# Autodesk Inventor assembly: Hand Assembly
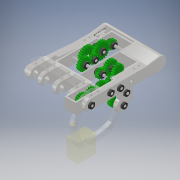
[picture p0: Inventor's stored thumbnail of the model, 180x180]
Saved by Autodesk Inventor 2017 (Build 210142000, 142)
## iProperties
Created: 2016-09-28
Part Number: Hand Assembly
Document SubType Name: Assembly
Designer: cmcdona
Author: cmcdona
## Documents named in this file (25)
- C:\Users\Sam\Desktop\1C03-20171130T033242Z-001\1C03\Project Files Final I Hope Maybe Not Probably Not\Hand Assembly.iam
- C:\Users\Sam\Desktop\1C03-20171130T033242Z-001\1C03\Project Files Final I Hope Maybe Not Probably Not\Hand - Frame.ipt
- C:\Users\Sam\Desktop\1C03-20171130T033242Z-001\1C03\Project Files Final I Hope Maybe Not Probably Not\Hand - Digit 4.ipt
- C:\Users\Sam\Desktop\1C03-20171130T033242Z-001\1C03\Project Files Final I Hope Maybe Not Probably Not\Hand - Digit 0-1.ipt
- C:\Users\Sam\Desktop\1C03-20171130T033242Z-001\1C03\Project Files Final I Hope Maybe Not Probably Not\Hand - Distal Bridge.ipt
- C:\Users\Sam\Desktop\1C03-20171130T033242Z-001\1C03\Project Files Final I Hope Maybe Not Probably Not\Hand - Digit 2-3.ipt
- C:\Users\Sam\Desktop\1C03-20171130T033242Z-001\1C03\Project Files Final I Hope Maybe Not Probably Not\Hand - Proximal Bridge.ipt
- C:\Users\Sam\Desktop\1C03-20171130T033242Z-001\1C03\Project Files Final I Hope Maybe Not Probably Not\Hand - Functional Workspace.ipt
- C:\Users\Sam\Desktop\1C03-20171130T033242Z-001\1C03\Project Files Final I Hope Maybe Not Probably Not\Input Motor.ipt
- C:\Users\Sam\Desktop\1C03-20171130T033242Z-001\1C03\Project Files\GIVEN PARTS\THREADED STUDS\91565A838_STEEL THREADED ROD.ipt
- C:\Users\Sam\Desktop\1C03-20171130T033242Z-001\1C03\Project Files\GIVEN PARTS\NUTS\90480A009_STEEL HEX NUT.ipt
- C:\Users\Sam\Desktop\1C03-20171130T033242Z-001\1C03\Project Files Final I Hope Maybe Not Probably Not\Hand Assembly\Design Accelerator\Spur Gears1.iam
- C:\Users\Sam\Desktop\1C03-20171130T033242Z-001\1C03\Project Files Final I Hope Maybe Not Probably Not\Hand Assembly\Design Accelerator\Spur Gears2.iam
- C:\Users\Sam\Desktop\1C03-20171130T033242Z-001\1C03\Project Files Final I Hope Maybe Not Probably Not\Hand Assembly\Design Accelerator\Spur Gear12.ipt
- C:\Users\Sam\Desktop\1C03-20171130T033242Z-001\1C03\Project Files\GIVEN PARTS\THREADED STUDS\91565A838_STEEL THREADED ROD FULL.ipt
- C:\Users\Sam\Desktop\1C03-20171130T033242Z-001\1C03\Project Files Final I Hope Maybe Not Probably Not\Hand Assembly\Design Accelerator\Spur Gears3.iam
- C:\Users\Sam\Desktop\1C03-20171130T033242Z-001\1C03\Project Files Final I Hope Maybe Not Probably Not\Hand Assembly\Design Accelerator\Spur Gears4.iam
- C:\Users\Sam\Desktop\1C03-20171130T033242Z-001\1C03\Project Files Final I Hope Maybe Not Probably Not\Hand Assembly\Design Accelerator\Spur Gears5.iam
- C:\Users\Sam\Desktop\1C03-20171130T033242Z-001\1C03\Project Files Final I Hope Maybe Not Probably Not\Midsection.ipt
- C:\Users\Sam\Desktop\1C03-20171130T033242Z-001\1C03\Project Files\GIVEN PARTS\THREADED STUDS\91565A838_STEEL THREADED ROD HALF.ipt
- C:\Users\Sam\Desktop\1C03-20171130T033242Z-001\1C03\Project Files Final I Hope Maybe Not Probably Not\Hand Assembly\Design Accelerator\Spur Gears6.iam
- C:\Users\Sam\Desktop\1C03-20171130T033242Z-001\1C03\Project Files\GIVEN PARTS\THREADED STUDS\91565A838_STEEL THREADED ROD FINAL.ipt
- C:\Users\Sam\Desktop\1C03-20171130T033242Z-001\1C03\Project Files Final I Hope Maybe Not Probably Not\Hand Assembly\Design Accelerator\Spur Gears7.iam
- C:\Users\Sam\Desktop\1C03-20171130T033242Z-001\1C03\Project Files\GIVEN PARTS\THREADED STUDS\Finger.ipt
- C:\Users\Sam\Desktop\Inventor Files\Version I\SENGH IS KENGH.ipt
## Components (58 placed, 18 different names)
1. SENGH IS KENGH:1 — Flush:45
2. Midsection:1 — Mate:68, Mate:69, Mate:70, Flush:41, Mate:75, Mate:83, Flush:45
3. Finger:4 — Mate:99, Flush:44
4. Finger:3 — Mate:96, Mate:98, Mate:99, Flush:44
5. Finger:2 — Flush:43, Mate:95
6. Finger:1 — Mate:89, Mate:91, Mate:93, Flush:43
7. Input Motor:1 — Mate:22, Mate:23, Mate:48, Mate:49, Mate:51
8. Hand - Functional Workspace:1 — Mate:19, Mate:20, Mate:21
9. Hand - Proximal Bridge:1 — Mate:16, Mate:17, Mate:18
10. Hand - Digit 2-3:3 — Mate:13, Mate:14, Mate:15, Mate:24, Mate:28
11. Hand - Digit 2-3:2 — Mate:10, Mate:11, Mate:12, Mate:69
12. Hand - Digit 2-3:1 — Mate:7, Mate:8, Mate:9
13. Hand - Distal Bridge:1 — Mate:4, Mate:5, Mate:6, Mate:7, Mate:8, Mate:9, Mate:10, Mate:11, Mate:12, Mate:13, Mate:14, Mate:15
14. Hand - Digit 0-1:1 — Mate:2, Flush:3, Mate:3, Mate:6, Mate:19, Mate:20, Mate:21, Mate:26, Mate:29, Mate:31, Mate:33, Mate:98
15. Hand - Digit 4:1 — Flush:1, Flush:2, Mate:1, Mate:4, Mate:5
16. Hand - Frame:1 — Flush:1, Flush:2, Mate:1, Mate:2, Flush:3, Mate:3, Mate:16, Mate:17, Mate:18, Mate:22, Mate:23, Mate:65, Mate:68, Mate:70, Flush:41, Mate:72, Mate:85
17. Spur Gears:4 [sub-assembly] — Mate:50, Mate:51, Mate:54, Mate:55, Mate:56, Mate:57, Mate:61
18. Spur Gears:5 [sub-assembly] — Mate:60, Mate:61, Mate:62, Mate:64, Mate:73
19. Spur Gears:6 [sub-assembly] — Mate:66, Mate:67, Mate:71, Insert:6, Insert:7
20. Spur Gear1:1 — Mate:34, Flush:8
21. Spur Gears:3 [sub-assembly] — Flush:39, Mate:39, Mate:40, Mate:43, Mate:44, Mate:45, Mate:46, Mate:86
22. Spur Gears:2 [sub-assembly] — Mate:32, Mate:33, Flush:8, Mate:40, Mate:41, Mate:42
23. Spur Gears:1 [sub-assembly] — Mate:27, Mate:28, Flush:39, Mate:39, Mate:91
24. Spur Gears:7 [sub-assembly] — Mate:74, Mate:75, Mate:77, Mate:79, Mate:81, Insert:8, Insert:9
25. Spur Gears:8 [sub-assembly] — Mate:84, Mate:85, Mate:86, Mate:87
26. 91565A838_STEEL THREADED ROD FULL:2 — Mate:48, Mate:49, Mate:50, Mate:52, Mate:53
27. 91565A838_STEEL THREADED ROD HALF:1 — Mate:71, Mate:72, Mate:74, Mate:76, Mate:78
28. 91565A838_STEEL THREADED ROD FINAL:1 — Mate:81, Mate:83, Mate:84, Mate:88
29. 91565A838_STEEL THREADED ROD:4 — Mate:44, Insert:11
30. 91565A838_STEEL THREADED ROD:1 — Mate:24, Mate:25, Flush:4, Mate:27, Insert:13, Mate:90
31. 91565A838_STEEL THREADED ROD:2 — Mate:29, Flush:6, Mate:30, Mate:32, Mate:34, Insert:2, Mate:97
32. 91565A838_STEEL THREADED ROD:3 — Insert:1, Mate:42, Insert:12
33. 91565A838_STEEL THREADED ROD:7 — Mate:45, Mate:47, Flush:42, Insert:10
34. 91565A838_STEEL THREADED ROD:5 — Mate:56, Insert:4, Mate:58, Mate:60
35. 91565A838_STEEL THREADED ROD:6 — Mate:64, Mate:65, Mate:66
36. 90480A009_STEEL HEX NUT:2 — Flush:7, Mate:30, Mate:31
37. 90480A009_STEEL HEX NUT:21 — Insert:12
38. 90480A009_STEEL HEX NUT:1 — Mate:25, Flush:5, Mate:26
39. 90480A009_STEEL HEX NUT:3 — Insert:2
40. 90480A009_STEEL HEX NUT:4 — Insert:1, Mate:41
41. 90480A009_STEEL HEX NUT:5 — Mate:46, Mate:47, Flush:42
42. 90480A009_STEEL HEX NUT:6 — Mate:43
43. 90480A009_STEEL HEX NUT:7 — Mate:52, Mate:55
44. 90480A009_STEEL HEX NUT:8 — Mate:53, Mate:54
45. 90480A009_STEEL HEX NUT:9 — Insert:4, Mate:57
46. 90480A009_STEEL HEX NUT:10 — Mate:58, Mate:62
47. 90480A009_STEEL HEX NUT:12 — Mate:73
48. 90480A009_STEEL HEX NUT:11 — Mate:67
49. 90480A009_STEEL HEX NUT:13 — Insert:6
50. 90480A009_STEEL HEX NUT:14 — Insert:7
51. 90480A009_STEEL HEX NUT:15 — Mate:76, Mate:77
52. 90480A009_STEEL HEX NUT:16 — Mate:78, Mate:79
53. 90480A009_STEEL HEX NUT:17 — Insert:8
54. 90480A009_STEEL HEX NUT:18 — Insert:9
55. 90480A009_STEEL HEX NUT:19 — Mate:87, Mate:88
56. 90480A009_STEEL HEX NUT:20 — Insert:10
57. 90480A009_STEEL HEX NUT:22 — Insert:11
58. 90480A009_STEEL HEX NUT:23 — Insert:13
## Relationships (118: Mate 91, Flush 14, Insert 13)
- Flush:1: Hand - Digit 4:1 ↔ Hand - Frame:1
- Flush:2: Hand - Digit 4:1 ↔ Hand - Frame:1
- Mate:1: Hand - Digit 4:1 ↔ Hand - Frame:1
- Mate:2: Hand - Digit 0-1:1 ↔ Hand - Frame:1
- Flush:3: Hand - Digit 0-1:1 ↔ Hand - Frame:1
- Mate:3: Hand - Digit 0-1:1 ↔ Hand - Frame:1
- Mate:4: Hand - Distal Bridge:1 ↔ Hand - Digit 4:1
- Mate:5: Hand - Distal Bridge:1 ↔ Hand - Digit 4:1
- Mate:6: Hand - Distal Bridge:1 ↔ Hand - Digit 0-1:1
- Mate:7: Hand - Digit 2-3:1 ↔ Hand - Distal Bridge:1
- Mate:8: Hand - Digit 2-3:1 ↔ Hand - Distal Bridge:1
- Mate:9: Hand - Digit 2-3:1 ↔ Hand - Distal Bridge:1
- Mate:10: Hand - Digit 2-3:2 ↔ Hand - Distal Bridge:1
- Mate:11: Hand - Digit 2-3:2 ↔ Hand - Distal Bridge:1
- Mate:12: Hand - Digit 2-3:2 ↔ Hand - Distal Bridge:1
- Mate:13: Hand - Digit 2-3:3 ↔ Hand - Distal Bridge:1
- Mate:14: Hand - Digit 2-3:3 ↔ Hand - Distal Bridge:1
- Mate:15: Hand - Digit 2-3:3 ↔ Hand - Distal Bridge:1
- Mate:16: Hand - Proximal Bridge:1 ↔ Hand - Frame:1
- Mate:17: Hand - Proximal Bridge:1 ↔ Hand - Frame:1
- Mate:18: Hand - Proximal Bridge:1 ↔ Hand - Frame:1
- Mate:19: Hand - Functional Workspace:1 ↔ Hand - Digit 0-1:1
- Mate:20 (41 mm): Hand - Functional Workspace:1 ↔ Hand - Digit 0-1:1
- Mate:21 (33 mm): Hand - Functional Workspace:1 ↔ Hand - Digit 0-1:1
- Mate:22: Input Motor:1 ↔ Hand - Frame:1
- Mate:23: Input Motor:1 ↔ Hand - Frame:1
- Mate:24: Hand - Digit 2-3:3 ↔ 91565A838_STEEL THREADED ROD:1
- Mate:25: 91565A838_STEEL THREADED ROD:1 ↔ 90480A009_STEEL HEX NUT:1
- Flush:4 (-0.5 mm): 91565A838_STEEL THREADED ROD:1
- Flush:5: 90480A009_STEEL HEX NUT:1
- Mate:26: Hand - Digit 0-1:1 ↔ 90480A009_STEEL HEX NUT:1
- Mate:27: Spur Gears:1 ↔ 91565A838_STEEL THREADED ROD:1
- Mate:28 (6.5 mm): Hand - Digit 2-3:3 ↔ Spur Gears:1
- Mate:29: Hand - Digit 0-1:1 ↔ 91565A838_STEEL THREADED ROD:2
- Flush:6 (-0.5 mm): 91565A838_STEEL THREADED ROD:2
- Flush:7: 90480A009_STEEL HEX NUT:2
- Mate:30: 91565A838_STEEL THREADED ROD:2 ↔ 90480A009_STEEL HEX NUT:2
- Mate:31: Hand - Digit 0-1:1 ↔ 90480A009_STEEL HEX NUT:2
- Mate:32: Spur Gears:2 ↔ 91565A838_STEEL THREADED ROD:2
- Mate:33 (6.5 mm): Hand - Digit 0-1:1 ↔ Spur Gears:2
- Mate:34: Spur Gear1:1 ↔ 91565A838_STEEL THREADED ROD:2
- Flush:8: Spur Gear1:1 ↔ Spur Gears:2
- Flush:39: Spur Gears:3 ↔ Spur Gears:1
- Mate:39 (16 mm): Spur Gears:3 ↔ Spur Gears:1
- Mate:40 (16 mm): Spur Gears:3 ↔ Spur Gears:2
- Insert:1 (-0.7 mm): 91565A838_STEEL THREADED ROD:3 ↔ 90480A009_STEEL HEX NUT:4
- Mate:41: Spur Gears:2 ↔ 90480A009_STEEL HEX NUT:4
- Mate:42: Spur Gears:2 ↔ 91565A838_STEEL THREADED ROD:3
- Insert:2 (0.7 mm): 91565A838_STEEL THREADED ROD:2 ↔ 90480A009_STEEL HEX NUT:3
- [Insert] (-0.7 mm): 91565A838_STEEL THREADED ROD:4 ↔ 90480A009_STEEL HEX NUT:6
- Mate:43: Spur Gears:3 ↔ 90480A009_STEEL HEX NUT:6
- Mate:44: Spur Gears:3 ↔ 91565A838_STEEL THREADED ROD:4
- Mate:45: Spur Gears:3 ↔ 91565A838_STEEL THREADED ROD:7
- Mate:46: Spur Gears:3 ↔ 90480A009_STEEL HEX NUT:5
- Mate:47: 91565A838_STEEL THREADED ROD:7 ↔ 90480A009_STEEL HEX NUT:5
- Mate:48: Input Motor:1 ↔ 91565A838_STEEL THREADED ROD FULL:2
- Mate:49: Input Motor:1 ↔ 91565A838_STEEL THREADED ROD FULL:2
- Mate:50: Spur Gears:4 ↔ 91565A838_STEEL THREADED ROD FULL:2
- Mate:51 (10 mm): Input Motor:1 ↔ Spur Gears:4
- Mate:52: 91565A838_STEEL THREADED ROD FULL:2 ↔ 90480A009_STEEL HEX NUT:7
- Mate:53: 91565A838_STEEL THREADED ROD FULL:2 ↔ 90480A009_STEEL HEX NUT:8
- Mate:54: Spur Gears:4 ↔ 90480A009_STEEL HEX NUT:8
- Mate:55: Spur Gears:4 ↔ 90480A009_STEEL HEX NUT:7
- Mate:56: Spur Gears:4 ↔ 91565A838_STEEL THREADED ROD:5
- Insert:4 (0.7 mm): 91565A838_STEEL THREADED ROD:5 ↔ 90480A009_STEEL HEX NUT:9
- Mate:57: Spur Gears:4 ↔ 90480A009_STEEL HEX NUT:9
- Mate:58: 91565A838_STEEL THREADED ROD:5 ↔ 90480A009_STEEL HEX NUT:10
- Mate:60: Spur Gears:5 ↔ 91565A838_STEEL THREADED ROD:5
- Mate:61: Spur Gears:4 ↔ Spur Gears:5
- Mate:62: Spur Gears:5 ↔ 90480A009_STEEL HEX NUT:10
- [Insert] (0.07 mm): 91565A838_STEEL THREADED ROD:6 ↔ 90480A009_STEEL HEX NUT:11
- [Mate]: 91565A838_STEEL THREADED ROD:6 ↔ 90480A009_STEEL HEX NUT:12
- Mate:64: Spur Gears:5 ↔ 91565A838_STEEL THREADED ROD:6
- Mate:65: Hand - Frame:1 ↔ 91565A838_STEEL THREADED ROD:6
- Mate:66: Spur Gears:6 ↔ 91565A838_STEEL THREADED ROD:6
- Mate:67: Spur Gears:6 ↔ 90480A009_STEEL HEX NUT:11
- Mate:68: Midsection:1 ↔ Hand - Frame:1
- Mate:69: Midsection:1 ↔ Hand - Digit 2-3:2
- Mate:70: Midsection:1 ↔ Hand - Frame:1
- Flush:41: Midsection:1 ↔ Hand - Frame:1
- Mate:71: Spur Gears:6 ↔ 91565A838_STEEL THREADED ROD HALF:1
- Mate:72 (-1.5 mm): Hand - Frame:1 ↔ 91565A838_STEEL THREADED ROD HALF:1
- Mate:73: Spur Gears:5 ↔ 90480A009_STEEL HEX NUT:12
- Insert:6: Spur Gears:6 ↔ 90480A009_STEEL HEX NUT:13
- Insert:7: Spur Gears:6 ↔ 90480A009_STEEL HEX NUT:14
- Flush:42 (0.7 mm): 91565A838_STEEL THREADED ROD:7 ↔ 90480A009_STEEL HEX NUT:5
- Mate:74: Spur Gears:7 ↔ 91565A838_STEEL THREADED ROD HALF:1
- Mate:75 (3.3 mm): Midsection:1 ↔ Spur Gears:7
- Mate:76: 91565A838_STEEL THREADED ROD HALF:1 ↔ 90480A009_STEEL HEX NUT:15
- Mate:77: Spur Gears:7 ↔ 90480A009_STEEL HEX NUT:15
- Mate:78: 91565A838_STEEL THREADED ROD HALF:1 ↔ 90480A009_STEEL HEX NUT:16
- Mate:79: Spur Gears:7 ↔ 90480A009_STEEL HEX NUT:16
- Mate:81: Spur Gears:7 ↔ 91565A838_STEEL THREADED ROD FINAL:1
- Mate:83: Midsection:1 ↔ 91565A838_STEEL THREADED ROD FINAL:1
- Insert:8: Spur Gears:7 ↔ 90480A009_STEEL HEX NUT:17
- Insert:9: Spur Gears:7 ↔ 90480A009_STEEL HEX NUT:18
- Mate:84: Spur Gears:8 ↔ 91565A838_STEEL THREADED ROD FINAL:1
- Mate:85 (0.5 mm): Hand - Frame:1 ↔ Spur Gears:8
- Mate:86 (16 mm): Spur Gears:3 ↔ Spur Gears:8
- Mate:87: Spur Gears:8 ↔ 90480A009_STEEL HEX NUT:19
- Mate:88: 91565A838_STEEL THREADED ROD FINAL:1 ↔ 90480A009_STEEL HEX NUT:19
- Insert:10 (0.5 mm): 91565A838_STEEL THREADED ROD:7 ↔ 90480A009_STEEL HEX NUT:20
- Insert:11 (0.5 mm): 91565A838_STEEL THREADED ROD:4 ↔ 90480A009_STEEL HEX NUT:22
- Insert:12 (0.5 mm): 91565A838_STEEL THREADED ROD:3 ↔ 90480A009_STEEL HEX NUT:21
- Insert:13 (0.7 mm): 91565A838_STEEL THREADED ROD:1 ↔ 90480A009_STEEL HEX NUT:23
- Mate:89: Finger:1
- Mate:90: 91565A838_STEEL THREADED ROD:1
- Mate:91: Finger:1 ↔ Spur Gears:1
- Mate:93: Finger:1
- Mate:94
- Flush:43: Finger:2 ↔ Finger:1
- Mate:95: Finger:2
- Mate:96: Finger:3
- Mate:97: 91565A838_STEEL THREADED ROD:2
- Mate:98: Finger:3 ↔ Hand - Digit 0-1:1
- Mate:99: Finger:4 ↔ Finger:3
- Flush:44: Finger:4 ↔ Finger:3
- Flush:45: SENGH IS KENGH:1 ↔ Midsection:1
## Named parameters: d54_d50 = -0.7 mm, d78_d70 = 0.07 mm, d79_d72 = 0 mm
